# Autodesk Inventor assembly: assembly
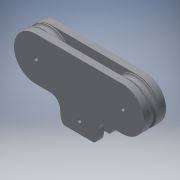
[picture p0: Inventor's stored thumbnail of the model, 180x180]
Saved by Autodesk Inventor 2016 (Build 200138000, 138)
## iProperties
Created: 2019-02-22
Part Number: assembly
Document SubType Name: Assembly
Designer: reesem783
Author: reesem783
## Documents named in this file (4)
- H:\Github\Zipline\Inventor\assembly.iam
- H:\Github\Zipline\Inventor\wheel.ipt
- H:\Github\Zipline\Inventor\casing.ipt
- H:\Github\Zipline\Inventor\bearing.ipt
## Components (8 placed, 3 different names)
1. casing:1 — Insert:1, Mate:1, Mate:2, Mate:10
2. casing:2 — Mate:9, Mate:10
3. bearing:1 — Mate:7, Mate:8
4. bearing:2 — Insert:1, Insert:2
5. bearing:3 — Mate:5, Mate:6, Mate:9
6. bearing:4 — Mate:1, Mate:2, Mate:3, Mate:4
7. wheel:1 — Insert:2, Mate:5, Mate:6
8. wheel:2 — Mate:3, Mate:4, Mate:7, Mate:8
## Relationships (12: Mate 10, Insert 2)
- Insert:1: casing:1 ↔ bearing:2
- Insert:2: bearing:2 ↔ wheel:1
- Mate:1: casing:1 ↔ bearing:4
- Mate:2: casing:1 ↔ bearing:4
- Mate:3: bearing:4 ↔ wheel:2
- Mate:4: bearing:4 ↔ wheel:2
- Mate:5: bearing:3 ↔ wheel:1
- Mate:6: bearing:3 ↔ wheel:1
- Mate:7: bearing:1 ↔ wheel:2
- Mate:8: bearing:1 ↔ wheel:2
- Mate:9: casing:2 ↔ bearing:3
- Mate:10: casing:1 ↔ casing:2
